# Autodesk Inventor assembly: DishFront
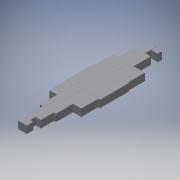
[picture p0: Inventor's stored thumbnail of the model, 180x180]
Saved by Autodesk Inventor 2016 (Build 200138000, 138)
## iProperties
Created: 2016-08-31
Part Number: DishFront
Document SubType Name: Assembly
Designer: jfixelle
Author: jfixelle
## Documents named in this file (7)
- E:\jfixelle\Documents\APC\GitRepo\FrontEnd\Placement\DishFront.iam
- E:\jfixelle\Documents\APC\GitRepo\FrontEnd\Placement\AmplifierBlock1.ipt
- E:\jfixelle\Documents\APC\GitRepo\FrontEnd\Placement\AmplifierBlock2.ipt
- E:\jfixelle\Documents\APC\GitRepo\FrontEnd\Placement\CombinerBlock.ipt
- E:\jfixelle\Documents\APC\GitRepo\FrontEnd\Placement\CouplerBlock.ipt
- E:\jfixelle\Documents\APC\GitRepo\FrontEnd\Placement\FilterBlock.ipt
- E:\jfixelle\Documents\APC\GitRepo\FrontEnd\Placement\UMCCBlock.ipt
## Components (16 placed, 6 different names)
1. AmplifierBlock1:1 — Flush:1, Flush:2, Flush:3, Flush:4, Flush:5, Flush:6
2. AmplifierBlock2:1 — Flush:14
3. CombinerBlock:1 — Flush:11
4. CouplerBlock:1 — Flush:9
5. FilterBlock:1 — Flush:4
6. UMCCBlock:1 — Flush:8
7. FilterBlock:2 — Flush:7
8. FilterBlock:3 — Flush:6
9. FilterBlock:4 — Flush:5
10. CombinerBlock:2 — Flush:1, Flush:7, Flush:8, Flush:9, Flush:10, Flush:11, Flush:12, Flush:13, Flush:14, Flush:15
11. CombinerBlock:3 — Flush:2
12. CombinerBlock:4 — Flush:3
13. CombinerBlock:5 — Flush:12
14. CombinerBlock:6 — Flush:13
15. UMCCBlock:2 — Flush:10
16. UMCCBlock:3 — Flush:15
## Relationships (15: Flush 15)
- Flush:1: AmplifierBlock1:1 ↔ CombinerBlock:2
- Flush:2: AmplifierBlock1:1 ↔ CombinerBlock:3
- Flush:3: AmplifierBlock1:1 ↔ CombinerBlock:4
- Flush:4: AmplifierBlock1:1 ↔ FilterBlock:1
- Flush:5: AmplifierBlock1:1 ↔ FilterBlock:4
- Flush:6: AmplifierBlock1:1 ↔ FilterBlock:3
- Flush:7: FilterBlock:2 ↔ CombinerBlock:2
- Flush:8: UMCCBlock:1 ↔ CombinerBlock:2
- Flush:9: CouplerBlock:1 ↔ CombinerBlock:2
- Flush:10: CombinerBlock:2 ↔ UMCCBlock:2
- Flush:11: CombinerBlock:1 ↔ CombinerBlock:2
- Flush:12: CombinerBlock:2 ↔ CombinerBlock:5
- Flush:13: CombinerBlock:2 ↔ CombinerBlock:6
- Flush:14: AmplifierBlock2:1 ↔ CombinerBlock:2
- Flush:15: CombinerBlock:2 ↔ UMCCBlock:3
